# Autodesk Inventor assembly: Front-Back Component Holds
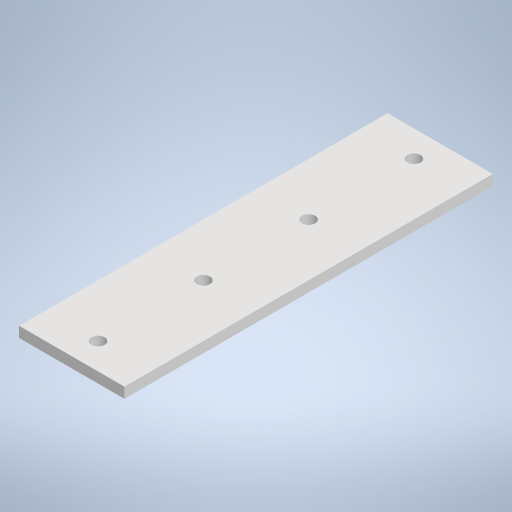
[picture p0: Inventor's stored thumbnail of the model, 512x512]
Saved by Autodesk Inventor 2024 (Build 280153000, 153)
## iProperties
Created: 2024-01-19
Part Number: Front-Back Component Holds
Document SubType Name: Assembly
Designer: Guru
Author: Guru
## Documents named in this file (2)
- D:\Project TRACER\Front-Back Component Holds.iam
- D:\Project TRACER\Chassis\Front-Back Sensor Holds.ipt
## Components (1 placed, 1 different names)
1. Front-Back Sensor Holds:1 — Mate:1, Mate:2, Mate:3
## Relationships (3: Mate 3)
- Mate:1: Front-Back Sensor Holds:1
- Mate:2: Front-Back Sensor Holds:1
- Mate:3: Front-Back Sensor Holds:1
